# Autodesk Inventor assembly: XEndRight
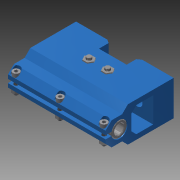
[picture p0: Inventor's stored thumbnail of the model, 180x180]
Saved by Autodesk Inventor 2015 SP1 (Build 190203100, 203)
## iProperties
Created: 2014-08-16
Part Number: XEndRight
Document SubType Name: Assembly
Designer: Jack
Mass: 125.348 g
Surface Area: 370.67 cm^2
Volume: 71.2484 cm^3
Density: 1.75931 g/cm^3
Author: Jack
Title: X End Right
## Documents named in this file (13)
- C:\Users\Jack\ownCloud\Projects\CrossBot\InventorModel\XAxis\XEndRight.iam
- C:\Users\Jack\ownCloud\Projects\CrossBot\InventorModel\Hardware\Nuts\Nut3.ipt
- C:\Users\Jack\ownCloud\Projects\CrossBot\InventorModel\Hardware\Bolts\SHCS\SHCS4\SHCS4x30.ipt
- C:\Users\Jack\ownCloud\Projects\CrossBot\InventorModel\Hardware\Nuts\Nut4.ipt
- C:\Users\Jack\ownCloud\Projects\CrossBot\InventorModel\Hardware\Bearing\BearingRadialBall\BearingRadialBallF624zz.ipt
- C:\Users\Jack\ownCloud\Projects\CrossBot\InventorModel\Hardware\Wahsers\M4Washer.ipt
- C:\Users\Jack\ownCloud\Projects\CrossBot\InventorModel\Hardware\Bolts\SHCS\SHCS3\SHCS3x8.ipt
- C:\Users\Jack\ownCloud\Projects\CrossBot\InventorModel\XAxis\XAxisBearingSpacer.ipt
- C:\Users\Jack\ownCloud\Projects\CrossBot\InventorModel\Hardware\Bearing\BearingLinear\BearingLinearLMK8.ipt
- C:\Users\Jack\ownCloud\Projects\CrossBot\InventorModel\Hardware\Belt\GT2Idler.iam
- C:\Users\Jack\ownCloud\Projects\CrossBot\InventorModel\XAxis\XAxisBeltIdlerSpacer.ipt
- C:\Users\Jack\ownCloud\Projects\CrossBot\InventorModel\XAxis\XEndRight.ipt
- C:\Users\Jack\ownCloud\Projects\CrossBot\InventorModel\Hardware\Bolts\SHCS\SHCS3\SHCS3x14.ipt
## Components (26 placed, 12 different names)
1. BearingLinearLMK8:1 — Mate:106, Flush:4
2. BearingLinearLMK8:2 — Mate:90, Flush:5
3. BearingRadialBallF624zz:1 — Mate:79, Mate:80, Mate:81, Mate:82
4. BearingRadialBallF624zz:2 — Mate:79, Mate:80, Mate:83
5. XAxisBearingSpacer:2 — Mate:84, Mate:85
6. GT2Idler:1 [sub-assembly] — Mate:86, Mate:121
7. XAxisBeltIdlerSpacer:1 — Mate:89, Mate:93, Mate:122
8. XEndRight:1 — Mate:90, Flush:3, Mate:91, Mate:92, Mate:94, Mate:95, Angle:1, Mate:96, Mate:97, Mate:98, Mate:99, Angle:2, Mate:100, Mate:101, Mate:102, Mate:103, Angle:3, Angle:4, Mate:104, Mate:105, Mate:106, Flush:4, Flush:5, Mate:109, Mate:110, Angle:5, Angle:6, Mate:112, Mate:113, Mate:115, Mate:116, Mate:118, Mate:119, Angle:7, Mate:120, Mate:122
9. M4Washer:4 — Mate:38, Mate:96
10. M4Washer:3 — Mate:65, Mate:93, Mate:121
11. M4Washer:2 — Mate:30, Mate:82, Mate:100
12. M4Washer:1 — Mate:64, Mate:83, Mate:85
13. Nut4:2 — Mate:21, Angle:2, Mate:101
14. Nut4:1 — Mate:20, Angle:1, Mate:97
15. SHCS4x30:2 — Mate:20, Mate:38, Mate:65, Mate:86, Mate:89, Mate:94, Mate:95
16. SHCS4x30:1 — Mate:21, Mate:30, Mate:64, Mate:81, Mate:84, Mate:98, Mate:99
17. Nut3:3 — Mate:43, Flush:1, Angle:4, Mate:104
18. Nut3:4 — Mate:42, Flush:2, Angle:3, Mate:105
19. SHCS3x8:1 — Mate:42, Flush:2, Mate:103
20. SHCS3x8:2 — Mate:43, Flush:1, Mate:102
21. SHCS3x14:2 — Mate:111, Mate:112, Mate:113
22. Nut3:2 — Mate:109, Angle:6, Mate:111
23. SHCS3x14:3 — Mate:118, Mate:120
24. Nut3:5 — Mate:119, Angle:7
25. SHCS3x14:1 — Mate:114, Mate:115, Mate:116
26. Nut3:1 — Mate:110, Angle:5, Mate:114
## Relationships (60: Mate 48, Angle 7, Flush 5)
- Mate:20: Nut4:1 ↔ SHCS4x30:2
- Mate:21: Nut4:2 ↔ SHCS4x30:1
- Mate:30: M4Washer:2 ↔ SHCS4x30:1
- Mate:38: M4Washer:4 ↔ SHCS4x30:2
- Mate:42: Nut3:4 ↔ SHCS3x8:1
- Mate:43: Nut3:3 ↔ SHCS3x8:2
- Flush:1 (-0.5 mm): Nut3:3 ↔ SHCS3x8:2
- Flush:2 (-0.5 mm): Nut3:4 ↔ SHCS3x8:1
- Mate:64: M4Washer:1 ↔ SHCS4x30:1
- Mate:65: M4Washer:3 ↔ SHCS4x30:2
- Mate:79: BearingRadialBallF624zz:1 ↔ BearingRadialBallF624zz:2
- Mate:80: BearingRadialBallF624zz:1 ↔ BearingRadialBallF624zz:2
- Mate:81: BearingRadialBallF624zz:1 ↔ SHCS4x30:1
- Mate:82: BearingRadialBallF624zz:1 ↔ M4Washer:2
- Mate:83: BearingRadialBallF624zz:2 ↔ M4Washer:1
- Mate:84: XAxisBearingSpacer:2 ↔ SHCS4x30:1
- Mate:85: XAxisBearingSpacer:2 ↔ M4Washer:1
- Mate:86: GT2Idler:1 ↔ SHCS4x30:2
- Mate:89: XAxisBeltIdlerSpacer:1 ↔ SHCS4x30:2
- Mate:90: BearingLinearLMK8:2 ↔ XEndRight:1
- Flush:3: XEndRight:1
- Mate:91: XEndRight:1
- Mate:92: XEndRight:1
- Mate:93: XAxisBeltIdlerSpacer:1 ↔ M4Washer:3
- Mate:94: XEndRight:1 ↔ SHCS4x30:2
- Mate:95: XEndRight:1 ↔ SHCS4x30:2
- Angle:1 (0 deg): XEndRight:1 ↔ Nut4:1
- Mate:96: XEndRight:1 ↔ M4Washer:4
- Mate:97: XEndRight:1 ↔ Nut4:1
- Mate:98: XEndRight:1 ↔ SHCS4x30:1
- Mate:99: XEndRight:1 ↔ SHCS4x30:1
- Angle:2 (0 deg): XEndRight:1 ↔ Nut4:2
- Mate:100: XEndRight:1 ↔ M4Washer:2
- Mate:101: XEndRight:1 ↔ Nut4:2
- Mate:102: XEndRight:1 ↔ SHCS3x8:2
- Mate:103: XEndRight:1 ↔ SHCS3x8:1
- Angle:3 (0 deg): XEndRight:1 ↔ Nut3:4
- Angle:4 (0 deg): XEndRight:1 ↔ Nut3:3
- Mate:104: XEndRight:1 ↔ Nut3:3
- Mate:105: XEndRight:1 ↔ Nut3:4
- Mate:106: BearingLinearLMK8:1 ↔ XEndRight:1
- Flush:4: BearingLinearLMK8:1 ↔ XEndRight:1
- Flush:5: BearingLinearLMK8:2 ↔ XEndRight:1
- Mate:109: XEndRight:1 ↔ Nut3:2
- Mate:110: XEndRight:1 ↔ Nut3:1
- Angle:5 (0 deg): XEndRight:1 ↔ Nut3:1
- Angle:6 (0 deg): XEndRight:1 ↔ Nut3:2
- Mate:111: SHCS3x14:2 ↔ Nut3:2
- Mate:112: XEndRight:1 ↔ SHCS3x14:2
- Mate:113: XEndRight:1 ↔ SHCS3x14:2
- Mate:114: SHCS3x14:1 ↔ Nut3:1
- Mate:115: XEndRight:1 ↔ SHCS3x14:1
- Mate:116: XEndRight:1 ↔ SHCS3x14:1
- [Mate]: SHCS3x14:3 ↔ Nut3:5
- Mate:118: XEndRight:1 ↔ SHCS3x14:3
- Mate:119: XEndRight:1 ↔ Nut3:5
- Angle:7 (0 deg): XEndRight:1 ↔ Nut3:5
- Mate:120: XEndRight:1 ↔ SHCS3x14:3
- Mate:121: GT2Idler:1 ↔ M4Washer:3
- Mate:122: XAxisBeltIdlerSpacer:1 ↔ XEndRight:1
## Named parameters: d161_d150 = 0 mm
